# Autodesk Inventor assembly: assy2
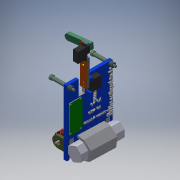
[picture p0: Inventor's stored thumbnail of the model, 180x180]
Saved by Autodesk Inventor 2018 (Build 220112000, 112)
## iProperties
Created: 2018-10-25
Part Number: assy2
Document SubType Name: Assembly
Designer: iki
Author: iki
## Documents named in this file (14)
- C:\Users\iki\Documents\Inventor\Crawler\assy2.iam
- C:\Users\iki\Documents\Inventor\Crawler\MainBody.ipt
- C:\Users\iki\Documents\Inventor\Crawler\servoMotor.ipt
- C:\Users\iki\Documents\Inventor\Crawler\Arm1.ipt
- C:\Users\iki\Documents\Inventor\Crawler\Arm2.ipt
- C:\Users\iki\Documents\Inventor\Crawler\Bearing Housing.ipt
- C:\Users\iki\Documents\Inventor\Crawler\Powerbank.ipt
- C:\Users\iki\Documents\Inventor\Crawler\RPI_Zero.ipt
- C:\Users\iki\Documents\Inventor\Crawler\Axel.ipt
- C:\Users\iki\Documents\Inventor\Crawler\Wheel.ipt
- C:\Users\iki\Documents\Inventor\Crawler\Encoder.ipt
- C:\Users\iki\Documents\Inventor\Crawler\leg_1.ipt
- C:\Users\iki\Documents\Inventor\Crawler\leg_2.ipt
- C:\Users\iki\Documents\Inventor\Crawler\BatteryHolder.ipt
## Components (18 placed, 13 different names)
1. MainBody:1 — Mate:1, Mate:2, Mate:3, Mate:5, Mate:11, Flush:1, Mate:12, Mate:13, Flush:2, Flush:3, Mate:14, Flush:4, Mate:15, Mate:16, Mate:17, Mate:25, Mate:26, Mate:28, Mate:29, Mate:30, Mate:32
2. servoMotor:1 — Mate:1, Mate:2, Mate:3, Mate:4
3. Arm1:1 — Mate:4, Mate:5, Mate:6, Mate:7, Mate:8, Mate:10
4. servoMotor:2 — Mate:6, Mate:7, Mate:8, Mate:9
5. Arm2:1 — Mate:9, Mate:10
6. Bearing Housing:1 — Mate:11, Flush:1, Mate:12, Mate:20
7. Bearing Housing:2 — Mate:13, Flush:2, Flush:3, Mate:18, Flush:5, Mate:22, Mate:23, Mate:24
8. Powerbank:1 — Mate:14, Flush:4
9. RPI_Zero:1 — Mate:15, Mate:16, Mate:17
10. Axel:1 — Mate:18, Flush:5, Mate:19, Mate:21
11. Wheel:1 — Mate:19, Mate:20
12. Wheel:2 — Mate:21, Mate:22
13. Encoder:1 — Mate:23, Mate:24
14. leg_1:1 — Mate:25, Mate:26, Mate:27
15. leg_2:1 — Mate:27, Mate:28
16. leg_1:2 — Mate:29, Mate:30, Mate:31
17. leg_2:2 — Mate:31, Mate:32
18. BatteryHolder:1
## Relationships (37: Mate 32, Flush 5)
- Mate:1: MainBody:1 ↔ servoMotor:1
- Mate:2: MainBody:1 ↔ servoMotor:1
- Mate:3: MainBody:1 ↔ servoMotor:1
- Mate:4: servoMotor:1 ↔ Arm1:1
- Mate:5 (3.5 mm): MainBody:1 ↔ Arm1:1
- Mate:6: Arm1:1 ↔ servoMotor:2
- Mate:7: Arm1:1 ↔ servoMotor:2
- Mate:8: Arm1:1 ↔ servoMotor:2
- Mate:9: servoMotor:2 ↔ Arm2:1
- Mate:10 (3.5 mm): Arm1:1 ↔ Arm2:1
- Mate:11: MainBody:1 ↔ Bearing Housing:1
- Flush:1 (8 mm): MainBody:1 ↔ Bearing Housing:1
- Mate:12 (-20 mm): MainBody:1 ↔ Bearing Housing:1
- Mate:13: MainBody:1 ↔ Bearing Housing:2
- Flush:2 (8 mm): MainBody:1 ↔ Bearing Housing:2
- Flush:3 (-7.5 mm): MainBody:1 ↔ Bearing Housing:2
- Mate:14: MainBody:1 ↔ Powerbank:1
- Flush:4 (2.5 mm): MainBody:1 ↔ Powerbank:1
- Mate:15: MainBody:1 ↔ RPI_Zero:1
- Mate:16: MainBody:1 ↔ RPI_Zero:1
- Mate:17: MainBody:1 ↔ RPI_Zero:1
- Mate:18: Bearing Housing:2 ↔ Axel:1
- Flush:5 (-5.5 mm): Bearing Housing:2 ↔ Axel:1
- Mate:19: Axel:1 ↔ Wheel:1
- Mate:20 (1.5 mm): Bearing Housing:1 ↔ Wheel:1
- Mate:21: Axel:1 ↔ Wheel:2
- Mate:22 (1.5 mm): Bearing Housing:2 ↔ Wheel:2
- Mate:23: Bearing Housing:2 ↔ Encoder:1
- Mate:24: Bearing Housing:2 ↔ Encoder:1
- Mate:25: MainBody:1 ↔ leg_1:1
- Mate:26: MainBody:1 ↔ leg_1:1
- Mate:27: leg_1:1 ↔ leg_2:1
- Mate:28: MainBody:1 ↔ leg_2:1
- Mate:29: MainBody:1 ↔ leg_1:2
- Mate:30: MainBody:1 ↔ leg_1:2
- Mate:31: leg_1:2 ↔ leg_2:2
- Mate:32: MainBody:1 ↔ leg_2:2
